# Autodesk Inventor assembly: gantry_frame
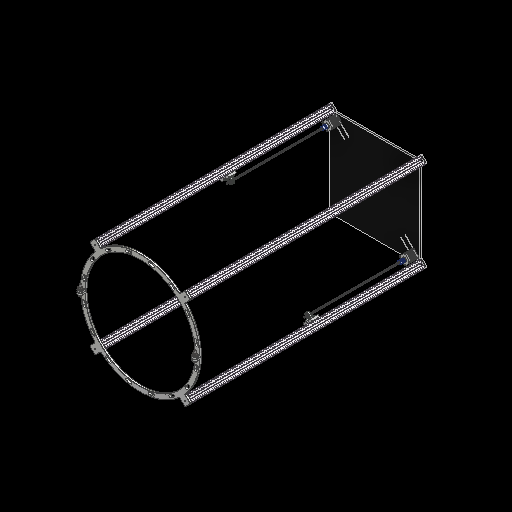
[picture p0: Inventor's stored thumbnail of the model, 512x512]
Saved by Autodesk Inventor 2026.1 (Build 301233000, 233)
## iProperties
Created: 2025-09-18
Part Number: gantry_frame
Document SubType Name: Assembly
Designer: drago
Author: drago
## Documents named in this file (6)
- C:\Users\drago\Desktop\_QIST4500_Multidisciplinary_Team_Project\Proteox MX magnet positioner CAD\gantry_frame.iam
- C:\Users\drago\Desktop\_QIST4500_Multidisciplinary_Team_Project\Proteox MX magnet positioner CAD\square_bar.ipt
- C:\Users\drago\Desktop\_QIST4500_Multidisciplinary_Team_Project\Proteox MX magnet positioner CAD\base_plate.ipt
- C:\Users\drago\Desktop\_QIST4500_Multidisciplinary_Team_Project\Proteox MX magnet positioner CAD\z_translator\z_Translator.iam
- C:\Users\drago\Desktop\_QIST4500_Multidisciplinary_Team_Project\Proteox MX magnet positioner CAD\full_ring.iam
- C:\Users\drago\Desktop\_QIST4500_Multidisciplinary_Team_Project\Proteox MX magnet positioner CAD\z_rail\Slider Assembly.iam
## Components (10 placed, 5 different names)
1. full_ring:1 [sub-assembly] — Mate:34, Mate:35, Mate:36, Mate:49
2. base_plate:1 — Mate:38, Angle:2, Mate:39, Mate:40, Mate:41, Mate:42, Mate:45, Mate:46, Mate:51, Mate:52, Mate:54, Mate:55
3. z_Translator:1 [sub-assembly] — Mate:41, Mate:44, Mate:46
4. z_Translator:2 [sub-assembly] — Mate:42, Mate:43, Mate:45
5. Slider Assembly:1 [sub-assembly] — Mate:50, Mate:51, Mate:52
6. Slider Assembly:2 [sub-assembly] — Mate:53, Mate:54, Mate:55
7. square_bar:1 — Mate:36, Angle:1, Mate:43
8. square_bar:2 — Mate:49, Mate:50
9. square_bar:3 — Mate:39, Mate:40, Mate:44
10. square_bar:4 — Mate:53
## Component patterns: (4 elements, first: square_bar:1)
## Relationships (21: Mate 19, Angle 2)
- Mate:34: full_ring:1
- Mate:35: full_ring:1
- Mate:36: full_ring:1 ↔ square_bar:1
- Angle:1 (45 deg): square_bar:1
- Mate:38: base_plate:1
- Angle:2 (45 deg): base_plate:1
- Mate:39: base_plate:1 ↔ square_bar:3
- Mate:40: base_plate:1 ↔ square_bar:3
- Mate:41: base_plate:1 ↔ z_Translator:1
- Mate:42: base_plate:1 ↔ z_Translator:2
- Mate:43: z_Translator:2 ↔ square_bar:1
- Mate:44: z_Translator:1 ↔ square_bar:3
- Mate:45: base_plate:1 ↔ z_Translator:2
- Mate:46: base_plate:1 ↔ z_Translator:1
- Mate:49: full_ring:1 ↔ square_bar:2
- Mate:50: Slider Assembly:1 ↔ square_bar:2
- Mate:51: base_plate:1 ↔ Slider Assembly:1
- Mate:52: base_plate:1 ↔ Slider Assembly:1
- Mate:53: Slider Assembly:2 ↔ square_bar:4
- Mate:54: base_plate:1 ↔ Slider Assembly:2
- Mate:55: base_plate:1 ↔ Slider Assembly:2
